# Autodesk Inventor assembly: test assembly
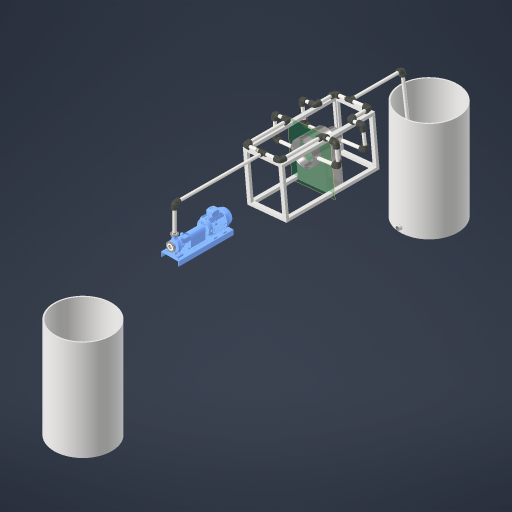
[picture p0: Inventor's stored thumbnail of the model, 512x512]
Saved by Autodesk Inventor 2023 (Build 270158000, 158)
## iProperties
Created: 2022-07-21
Part Number: test assembly
Document SubType Name: Assembly
Designer: station
Mass: 3659.88 g
Surface Area: 4755.26 cm^2
Volume: 455.583 cm^3
Density: 8.0334 g/cm^3
Author: station
## Documents named in this file (11)
- C:\Users\Mike\Desktop\Mechatronics\Mechatronics 5.1\Liquid-engine-cooling-system\design files\Ethanol engine 5 -inventor\test assembly.iam
- C:\Users\Mike\Desktop\Mechatronics\Mechatronics 5.1\Liquid-engine-cooling-system\design files\Ethanol engine 5 -inventor\inner wall.ipt
- C:\Users\Mike\Desktop\Mechatronics\Mechatronics 5.1\Liquid-engine-cooling-system\design files\Ethanol engine 5 -inventor\new outer wall.ipt
- C:\Users\Mike\Desktop\Mechatronics\Mechatronics 5.1\Liquid-engine-cooling-system\design files\Ethanol engine 5 -inventor\back bracket 2.ipt
- C:\Users\Mike\Desktop\Mechatronics\Mechatronics 5.1\Liquid-engine-cooling-system\design files\Ethanol engine 5 -inventor\back bracket.ipt
- C:\Users\Mike\Desktop\Mechatronics\Mechatronics 5.1\Liquid-engine-cooling-system\design files\Ethanol engine 5 -inventor\bracket 1.ipt
- C:\Users\Mike\Desktop\Mechatronics\Mechatronics 5.1\Liquid-engine-cooling-system\design files\Ethanol engine 5 -inventor\Support.ipt
- C:\Users\Mike\Desktop\Mechatronics\Mechatronics 5.1\Liquid-engine-cooling-system\design files\Ethanol engine 5 -inventor\Tank_M.ipt
- C:\Users\Mike\Desktop\Mechatronics\Mechatronics 5.1\Liquid-engine-cooling-system\design files\Ethanol engine 5 -inventor\test assembly\AIP\Tube and Pipe\test assembly.Tube and Pipe Runs.iam
- C:\Users\Mike\Desktop\Mechatronics\Mechatronics 5.1\Liquid-engine-cooling-system\centrifugal-pump-93.snapshot.8\Pump - KSB Etanorm 65-40-250 - emotor 180M.ipt
- C:\Users\Mike\Desktop\Mechatronics\Mechatronics 5.1\Liquid-engine-cooling-system\design files\Ethanol engine 5 -inventor\OuterShell.ipt
## Components (11 placed, 10 different names)
1. inner wall:1 — Mate:1, Flush:1, Mate:2, Mate:4
2. new outer wall:1 — Mate:1, Flush:1, Mate:3, Mate:5, Mate:6, Mate:7, Mate:12, Mate:13
3. back bracket 2:1 — Mate:2, Mate:3, Mate:8
4. back bracket:1 — Mate:4, Mate:5, Mate:8
5. bracket 1:1 — Mate:6, Mate:7
6. Support:1 — Mate:9, Mate:10, Mate:11, Mate:12, Mate:13
7. Tank_M:1 — Mate:14
8. Tank_M:2 — Mate:15
9. Tube & Pipe Runs [sub-assembly]
10. Pump - KSB Etanorm 65-40-250 - emotor 180M:1
11. OuterShell:1 — Mate:9, Mate:10, Mate:11, Mate:14, Mate:15
## Relationships (16: Mate 15, Flush 1)
- Mate:1: inner wall:1 ↔ new outer wall:1
- Flush:1: inner wall:1 ↔ new outer wall:1
- Mate:2: inner wall:1 ↔ back bracket 2:1
- Mate:3 (-14.601 mm): new outer wall:1 ↔ back bracket 2:1
- Mate:4: inner wall:1 ↔ back bracket:1
- Mate:5 (-3.601 mm): new outer wall:1 ↔ back bracket:1
- Mate:6: new outer wall:1 ↔ bracket 1:1
- Mate:7 (-18 mm): new outer wall:1 ↔ bracket 1:1
- Mate:8: back bracket 2:1 ↔ back bracket:1
- Mate:9: Support:1 ↔ OuterShell:1
- Mate:10: Support:1 ↔ OuterShell:1
- Mate:11 (190 mm): Support:1 ↔ OuterShell:1
- Mate:12: new outer wall:1 ↔ Support:1
- Mate:13: new outer wall:1 ↔ Support:1
- Mate:14 (-1580 mm): Tank_M:1 ↔ OuterShell:1
- Mate:15 (696 mm): Tank_M:2 ↔ OuterShell:1
